# Autodesk Inventor assembly: Arm for Gen 2
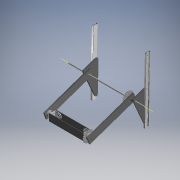
[picture p0: Inventor's stored thumbnail of the model, 180x180]
Saved by Autodesk Inventor 2019 (Build 230136000, 136)
## iProperties
Part Number: Arm for Gen 2
Document SubType Name: Assembly
Designer: Delta
Author: Delta
## Documents named in this file (11)
- C:\Robotics\2019-20_CAD\Collection\Arm for Gen 2.iam
- C:\Robotics\2019-20_CAD\Collection\12 Inch Hex Axle.ipt
- C:\Robotics\COTSParts\Sprockets - AndyMark\615106.ipt
- C:\Robotics\2019-20_CAD\Collection\bar arms.ipt
- C:\Robotics\2019-20_CAD\Collection\Claw holding bars.ipt
- C:\Robotics\COTSParts\Tetrix\39270_txm-insidecconnectors.ipt
- C:\Robotics\COTSParts\Actobotics\545 parts\545364 assembly.ipt
- C:\Robotics\COTSParts\Actobotics\545 parts\545456PatternAdapter.77in.625in.ipt
- C:\Robotics\2019-20_CAD\Collection\Spacer .25D .375H.ipt
- C:\Robotics\2019-20_CAD\Collection\Wing Left.iam
- C:\Robotics\2019-20_CAD\Collection\Wing Right.iam
## Components (17 placed, 10 different names)
1. 12 Inch Hex Axle:1 — Mate:5, Mate:6, Mate:8, Mate:52, Mate:55, Mate:57, Mate:59, Mate:61
2. 615106:1 — Mate:5, Mate:51
3. bar arms:1 — Mate:6, Flush:5, Mate:41, Mate:50, Mate:53
4. bar arms:2 — Mate:8, Flush:5, Mate:45, Mate:51, Mate:54, Mate:58
5. Claw holding bars:1 — Mate:22, Mate:23, Mate:24, Mate:25, Mate:26, Mate:27, Angle:2
6. 615106:2 — Mate:46, Mate:47, Mate:48, Mate:49
7. 39270_txm-insidecconnectors:1 — Mate:25, Mate:26, Mate:27, Mate:31, Mate:32
8. 39270_txm-insidecconnectors:2 — Mate:22, Mate:23, Mate:24, Mate:29, Mate:42, Mate:43
9. 545364 assembly:1 — Mate:33, Mate:35, Mate:45, Mate:47
10. 545364 assembly:2 — Mate:37, Mate:38, Mate:39, Mate:41, Mate:50
11. 545456PatternAdapter.77in.625in:1 — Mate:31, Mate:32, Mate:33, Mate:35, Mate:46, Mate:48, Mate:49
12. 545456PatternAdapter.77in.625in:2 — Mate:29, Mate:37, Mate:38, Mate:39, Mate:42, Mate:43
13. Spacer .25D .375H:1 — Mate:54, Mate:55
14. Spacer .25D .375H:2 — Mate:52, Mate:53, Mate:62
15. Spacer .25D .375H:3 — Mate:57, Mate:58, Mate:60
16. Wing Left:1 [sub-assembly] — Mate:61, Angle:1, Mate:62, Angle:2
17. Wing Right:1 [sub-assembly] — Mate:59, Mate:60, Angle:1
## Relationships (40: Mate 37, Angle 2, Flush 1)
- Mate:5: 12 Inch Hex Axle:1 ↔ 615106:1
- Mate:6: 12 Inch Hex Axle:1 ↔ bar arms:1
- Mate:8: 12 Inch Hex Axle:1 ↔ bar arms:2
- Flush:5: bar arms:1 ↔ bar arms:2
- Mate:22: Claw holding bars:1 ↔ 39270_txm-insidecconnectors:2
- Mate:23: Claw holding bars:1 ↔ 39270_txm-insidecconnectors:2
- Mate:24: Claw holding bars:1 ↔ 39270_txm-insidecconnectors:2
- Mate:25: Claw holding bars:1 ↔ 39270_txm-insidecconnectors:1
- Mate:26: Claw holding bars:1 ↔ 39270_txm-insidecconnectors:1
- Mate:27: Claw holding bars:1 ↔ 39270_txm-insidecconnectors:1
- Mate:29: 39270_txm-insidecconnectors:2 ↔ 545456PatternAdapter.77in.625in:2
- Mate:31: 39270_txm-insidecconnectors:1 ↔ 545456PatternAdapter.77in.625in:1
- Mate:32: 39270_txm-insidecconnectors:1 ↔ 545456PatternAdapter.77in.625in:1
- Mate:33: 545364 assembly:1 ↔ 545456PatternAdapter.77in.625in:1
- Mate:35: 545364 assembly:1 ↔ 545456PatternAdapter.77in.625in:1
- Mate:37: 545364 assembly:2 ↔ 545456PatternAdapter.77in.625in:2
- Mate:38: 545364 assembly:2 ↔ 545456PatternAdapter.77in.625in:2
- Mate:39: 545364 assembly:2 ↔ 545456PatternAdapter.77in.625in:2
- Mate:41: bar arms:1 ↔ 545364 assembly:2
- Mate:42: 39270_txm-insidecconnectors:2 ↔ 545456PatternAdapter.77in.625in:2
- Mate:43 (0.0762 mm): 39270_txm-insidecconnectors:2 ↔ 545456PatternAdapter.77in.625in:2
- Mate:45: bar arms:2 ↔ 545364 assembly:1
- Mate:46: 615106:2 ↔ 545456PatternAdapter.77in.625in:1
- Mate:47: 615106:2 ↔ 545364 assembly:1
- Mate:48: 615106:2 ↔ 545456PatternAdapter.77in.625in:1
- Mate:49: 615106:2 ↔ 545456PatternAdapter.77in.625in:1
- Mate:50: bar arms:1 ↔ 545364 assembly:2
- Mate:51 (9.6266 mm): 615106:1 ↔ bar arms:2
- Mate:52: 12 Inch Hex Axle:1 ↔ Spacer .25D .375H:2
- Mate:53: bar arms:1 ↔ Spacer .25D .375H:2
- Mate:54: bar arms:2 ↔ Spacer .25D .375H:1
- Mate:55: 12 Inch Hex Axle:1 ↔ Spacer .25D .375H:1
- Mate:57: 12 Inch Hex Axle:1 ↔ Spacer .25D .375H:3
- Mate:58: bar arms:2 ↔ Spacer .25D .375H:3
- Mate:59: 12 Inch Hex Axle:1 ↔ Wing Right:1
- Mate:60: Spacer .25D .375H:3 ↔ Wing Right:1
- Mate:61: 12 Inch Hex Axle:1 ↔ Wing Left:1
- Angle:1 (0 deg): Wing Left:1 ↔ Wing Right:1
- Mate:62: Spacer .25D .375H:2 ↔ Wing Left:1
- Angle:2 (0 deg): Claw holding bars:1 ↔ Wing Left:1
